# Autodesk Inventor assembly: Frame Long Side
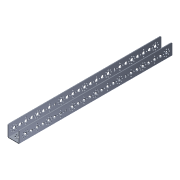
[picture p0: Inventor's stored thumbnail of the model, 180x180]
Saved by Autodesk Inventor 2015 (Build 190159000, 159)
## iProperties
Created: 2015-01-22
Part Number: Frame Long Side
Document SubType Name: Assembly
Designer: rihoobler
Author: rihoobler
## Documents named in this file (2)
- C:\Users\rihoobler\Documents\Inventor\SerenityMk.2\Frame Long Side.iam
- C:\Users\rihoobler\Documents\Inventor\SerenityMk.2\Imported Components\tetrix_739068_2012_288_channel\tetrix_739068_2012_288_channel.ipt
## Components (2 placed, 1 different names)
1. tetrix_739068_2012_288_channel:1 — Mate:1, Flush:1, Flush:2
2. tetrix_739068_2012_288_channel:2 — Mate:1, Flush:1, Flush:2
## Relationships (3: Flush 2, Mate 1)
- Mate:1: tetrix_739068_2012_288_channel:1 ↔ tetrix_739068_2012_288_channel:2
- Flush:1: tetrix_739068_2012_288_channel:1 ↔ tetrix_739068_2012_288_channel:2
- Flush:2: tetrix_739068_2012_288_channel:1 ↔ tetrix_739068_2012_288_channel:2
